# Autodesk Inventor assembly: ImpresionMotor
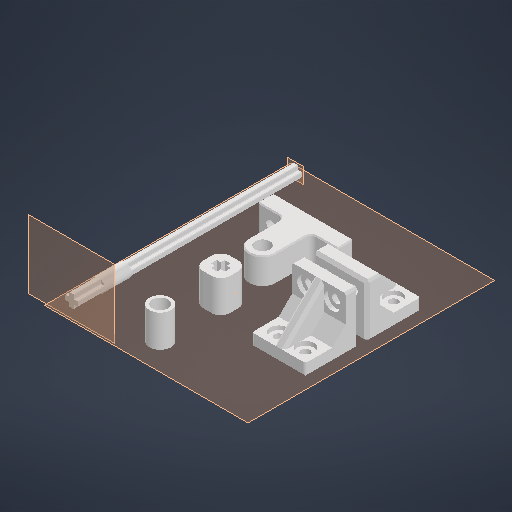
[picture p0: Inventor's stored thumbnail of the model, 512x512]
Saved by Autodesk Inventor 2026.3 (Build 303398000, 398)
## iProperties
Created: 2026-05-15
Part Number: ImpresionMotor
Document SubType Name: Assembly
Designer: Caro
Author: Caro
## Documents named in this file (6)
- C:\Users\Caro\JoseCarlos\TEC\TFG\Inventor\PiezasSTD\EnsamblesDeImpresion\ImpresionMotor.iam
- C:\Users\Caro\JoseCarlos\TEC\TFG\Inventor\PiezasSTD\Acoplador.ipt
- C:\Users\Caro\JoseCarlos\TEC\TFG\Inventor\PiezasSTD\EnsambleMotor\SoporteEjeMotor.ipt
- C:\Users\Caro\JoseCarlos\TEC\TFG\Inventor\PiezasSTD\EnsambleMotor\EjeDelMotor.ipt
- C:\Users\Caro\JoseCarlos\TEC\TFG\Inventor\PiezasSTD\EnsambleMotor\AcopleMotor.ipt
- C:\Users\Caro\JoseCarlos\TEC\TFG\Inventor\PiezasSTD\T.ipt
## Components (6 placed, 5 different names)
1. Acoplador:1 — Coincidencia:1
2. SoporteEjeMotor:1 — Coincidencia:2
3. EjeDelMotor:1 — Coincidencia:3
4. AcopleMotor:1 — Coincidencia:4
5. T:1 — Coincidencia:5, Ángulo:1
6. T:2 — Ángulo:1, Coincidencia:6
## Relationships (7: Mate 6, Angle 1)
- Coincidencia:1 [Mate]: Acoplador:1
- Coincidencia:2 [Mate]: SoporteEjeMotor:1
- Coincidencia:3 [Mate]: EjeDelMotor:1
- Coincidencia:4 [Mate]: AcopleMotor:1
- Coincidencia:5 [Mate]: T:1
- Ángulo:1 [Angle] (180 deg): T:1 ↔ T:2
- Coincidencia:6 [Mate]: T:2
